# Autodesk Inventor assembly: SRM rocket test stand
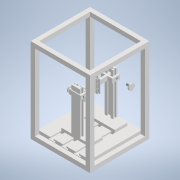
[picture p0: Inventor's stored thumbnail of the model, 180x180]
Saved by Autodesk Inventor 2022 (Build 260153000, 153)
## iProperties
Created: 2021-06-24
Part Number: SRM rocket test stand
Document SubType Name: Assembly
Designer: Admin
Author: Admin
## Documents named in this file (8)
- C:\Users\Admin\Documents\Inventor\SRM rocket test stand.iam
- C:\Users\Admin\Documents\Inventor\Frame.ipt
- C:\Users\Admin\Downloads\base plate.ipt
- C:\Users\Admin\Documents\Inventor\Clamp jaw handle.ipt
- C:\Users\Admin\Documents\Inventor\Clamp jaw.ipt
- C:\Users\Admin\Documents\Inventor\Clamp jaw handle_MIR.ipt
- C:\Users\Admin\Documents\Inventor\Clamp jaw_MIR.ipt
- C:\Users\Admin\Documents\Inventor\Knob.ipt
## Components (10 placed, 7 different names)
1. Frame:1 — Mate:1, Mate:2, Mate:3
2. base plate:1 — Mate:1, Mate:2, Mate:3, Mate:4, Mate:10, Mate:11, Mate:12, Mate:17
3. Clamp jaw handle:1 — Mate:4, Mate:6, Mate:7, Mate:17
4. Clamp jaw:1 — Mate:6, Mate:7, Mate:15, Mate:16
5. Clamp jaw handle_MIR:1 — Mate:8, Mate:9, Mate:10, Mate:11, Mate:12
6. Clamp jaw_MIR:1 — Mate:8, Mate:9, Mate:13, Mate:14
7. Knob:1 — Mate:16
8. Knob:2 — Mate:14
9. Knob:4 — Mate:13
10. Knob:5 — Mate:15
## Relationships (16: Mate 16)
- Mate:1: Frame:1 ↔ base plate:1
- Mate:2: Frame:1 ↔ base plate:1
- Mate:3: Frame:1 ↔ base plate:1
- Mate:4: base plate:1 ↔ Clamp jaw handle:1
- Mate:6: Clamp jaw handle:1 ↔ Clamp jaw:1
- Mate:7: Clamp jaw handle:1 ↔ Clamp jaw:1
- Mate:8: Clamp jaw handle_MIR:1 ↔ Clamp jaw_MIR:1
- Mate:9: Clamp jaw handle_MIR:1 ↔ Clamp jaw_MIR:1
- Mate:10: base plate:1 ↔ Clamp jaw handle_MIR:1
- Mate:11: base plate:1 ↔ Clamp jaw handle_MIR:1
- Mate:12: base plate:1 ↔ Clamp jaw handle_MIR:1
- Mate:13: Clamp jaw_MIR:1 ↔ Knob:4
- Mate:14: Clamp jaw_MIR:1 ↔ Knob:2
- Mate:15: Clamp jaw:1 ↔ Knob:5
- Mate:16: Clamp jaw:1 ↔ Knob:1
- Mate:17: base plate:1 ↔ Clamp jaw handle:1
